# Autodesk Inventor assembly: heater assembly_v5
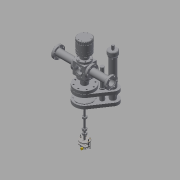
[picture p0: Inventor's stored thumbnail of the model, 180x180]
Saved by Autodesk Inventor 2019 (Build 230136000, 136)
## iProperties
Created: 2015-02-04
Part Number: heater assembly_v5
Document SubType Name: Assembly
Designer: Pascal
Author: Pascal
## Documents named in this file (13)
- C:\Users\user\Documents\Inventor@SVN\Moore Scienta DA30 system\e-beam-heater-Moore\heater assembly_v5.iam
- C:\Users\user\Documents\Inventor@SVN\Moore Scienta DA30 system\QMSC Heater_v3\rotary feedthrough (MDC 670024) length extension.ipt
- C:\Users\user\Documents\Inventor@SVN\Moore Scienta DA30 system\QMSC Heater_v3\9633T800_TWO-PIECE CLAMP-ON SHAFT COLLAR MOD.ipt
- C:\Users\user\Documents\Inventor@SVN\Moore Scienta DA30 system\QMSC Heater_v3\Ceramic eyelet.ipt
- C:\Users\user\Documents\Inventor@SVN\Moore Scienta DA30 system\QMSC Heater_v3\ANSI B18.2.2 - 6 - 32(06).ipt
- C:\Users\user\Documents\Inventor@SVN\Moore Scienta DA30 system\QMSC Heater_v3\MolyRodLong.ipt
- C:\Users\user\Documents\Inventor@SVN\Moore Scienta DA30 system\QMSC Heater_v3\BulletHolderAssembly.iam
- C:\Users\user\Documents\Inventor@SVN\Moore Scienta DA30 system\QMSC Heater_v3\MolyRodBulletPotential_v5.ipt
- C:\Users\user\Documents\Inventor@SVN\Moore Scienta DA30 system\QMSC Heater_v3\Shield_3_v5.ipt
- C:\Users\user\Documents\Inventor@SVN\Moore Scienta DA30 system\QMSC Heater_v3\2p75_6_way_cube_408001.ipt
- C:\Users\user\Documents\Inventor@SVN\Moore Scienta DA30 system\QMSC Heater_v3\4p5_to_2p75_reducer_402013.ipt
- C:\Users\user\Documents\Inventor@SVN\RM 479 ARPES and MOORE lab\diff_pump_stage\2p75_nipple_402002.ipt
- C:\Users\user\Documents\Inventor@SVN\Moore Scienta DA30 system\450LinearStage.iam
## Components (27 placed, 12 different names)
1. rotary feedthrough (MDC 670024) length extension:1 — Mate:45, Mate:47, Mate:49, Mate:53, Mate:111, Mate:162, Mate:171, Mate:182, Mate:183, Mate:190
2. 9633T800_TWO-PIECE CLAMP-ON SHAFT COLLAR MOD:1 — Mate:45, Mate:176, Mate:177
3. 9633T800_TWO-PIECE CLAMP-ON SHAFT COLLAR MOD:2 — Mate:49, Mate:50
4. 9633T800_TWO-PIECE CLAMP-ON SHAFT COLLAR MOD:3 — Mate:47, Mate:50
5. Shield_3_v5:1 — Mate:53, Mate:55, Mate:57, Mate:58, Mate:59, Mate:60, Mate:70, Mate:151, Mate:157, Mate:159, Mate:163, Mate:171, Mate:176, Mate:178, Mate:190
6. Ceramic eyelet:1 — Mate:55, Mate:155, Mate:156, Mate:157
7. Ceramic eyelet:2 — Mate:57, Mate:58, Mate:78, Mate:83, Mate:85
8. Ceramic eyelet:3 — Mate:59, Mate:60, Mate:61, Mate:62, Mate:63, Mate:64, Mate:161
9. Hex Machine Screw Nut - Inch 6 - 32:1 — Mate:61, Mate:62
10. Hex Machine Screw Nut - Inch 6 - 32:2 — Mate:63, Mate:64, Mate:174
11. Ceramic eyelet:7 — Mate:70, Flush:23, Mate:159, Mate:160
12. MolyRodBulletPotential_v5:1 — Mate:78, Mate:84, Mate:86, Flush:26, Mate:169
13. Hex Machine Screw Nut - Inch 6 - 32:3 — Mate:173, Mate:174, Mate:175
14. Hex Machine Screw Nut - Inch 6 - 32:4 — Mate:172, Mate:175
15. Hex Machine Screw Nut - Inch 6 - 32:5 — Mate:83, Mate:84
16. Hex Machine Screw Nut - Inch 6 - 32:6 — Mate:85, Mate:86
17. MolyRodBulletPotential_v5:2 — Mate:155, Mate:156, Flush:25, Mate:167
18. Hex Machine Screw Nut - Inch 6 - 32:7 — Mate:166, Mate:167
19. Hex Machine Screw Nut - Inch 6 - 32:8 — Mate:168, Mate:169
20. MolyRodLong:1 — Flush:24, Mate:160
21. MolyRodLong:2 — Flush:23, Flush:24, Mate:161, Mate:172, Mate:173
22. BulletHolderAssembly:1 [sub-assembly] — Mate:151, Flush:25, Flush:26, Mate:166, Mate:168, Mate:178, Mate:179, Angle:1
23. 2p75_6_way_cube_408001:1 — Mate:182, Mate:183, Mate:184, Mate:185, Mate:186, Mate:187
24. 4p5_to_2p75_reducer_402013:1 — Mate:188, Mate:189
25. 2p75_nipple_402002:1 — Mate:184, Mate:185
26. 2p75_nipple_402002:2 — Mate:186, Mate:187, Angle:1
27. 450LinearStage:1 [sub-assembly] — Mate:188, Mate:189
## Relationships (59: Mate 54, Flush 4, Angle 1)
- Mate:45: rotary feedthrough (MDC 670024) length extension:1 ↔ 9633T800_TWO-PIECE CLAMP-ON SHAFT COLLAR MOD:1
- Mate:47: rotary feedthrough (MDC 670024) length extension:1 ↔ 9633T800_TWO-PIECE CLAMP-ON SHAFT COLLAR MOD:3
- Mate:49: rotary feedthrough (MDC 670024) length extension:1 ↔ 9633T800_TWO-PIECE CLAMP-ON SHAFT COLLAR MOD:2
- Mate:50 (50.8 mm): 9633T800_TWO-PIECE CLAMP-ON SHAFT COLLAR MOD:2 ↔ 9633T800_TWO-PIECE CLAMP-ON SHAFT COLLAR MOD:3
- Mate:53: rotary feedthrough (MDC 670024) length extension:1 ↔ Shield_3_v5:1
- Mate:55: Shield_3_v5:1 ↔ Ceramic eyelet:1
- Mate:57: Shield_3_v5:1 ↔ Ceramic eyelet:2
- Mate:58: Shield_3_v5:1 ↔ Ceramic eyelet:2
- Mate:59: Shield_3_v5:1 ↔ Ceramic eyelet:3
- Mate:60: Shield_3_v5:1 ↔ Ceramic eyelet:3
- Mate:61: Ceramic eyelet:3 ↔ Hex Machine Screw Nut - Inch 6 - 32:1
- Mate:62: Ceramic eyelet:3 ↔ Hex Machine Screw Nut - Inch 6 - 32:1
- Mate:63: Ceramic eyelet:3 ↔ Hex Machine Screw Nut - Inch 6 - 32:2
- Mate:64: Ceramic eyelet:3 ↔ Hex Machine Screw Nut - Inch 6 - 32:2
- Mate:70: Shield_3_v5:1 ↔ Ceramic eyelet:7
- Mate:78: Ceramic eyelet:2 ↔ MolyRodBulletPotential_v5:1
- Mate:83: Ceramic eyelet:2 ↔ Hex Machine Screw Nut - Inch 6 - 32:5
- Mate:84: MolyRodBulletPotential_v5:1 ↔ Hex Machine Screw Nut - Inch 6 - 32:5
- Mate:85: Ceramic eyelet:2 ↔ Hex Machine Screw Nut - Inch 6 - 32:6
- Mate:86: MolyRodBulletPotential_v5:1 ↔ Hex Machine Screw Nut - Inch 6 - 32:6
- Flush:23 (-5.08 mm): Ceramic eyelet:7 ↔ MolyRodLong:2
- Flush:24: MolyRodLong:1 ↔ MolyRodLong:2
- Mate:111: rotary feedthrough (MDC 670024) length extension:1
- Mate:151 (19.05 mm): Shield_3_v5:1 ↔ BulletHolderAssembly:1
- Mate:155: Ceramic eyelet:1 ↔ MolyRodBulletPotential_v5:2
- Mate:156: Ceramic eyelet:1 ↔ MolyRodBulletPotential_v5:2
- Mate:157: Shield_3_v5:1 ↔ Ceramic eyelet:1
- Mate:159: Shield_3_v5:1 ↔ Ceramic eyelet:7
- Mate:160: Ceramic eyelet:7 ↔ MolyRodLong:1
- Mate:161: Ceramic eyelet:3 ↔ MolyRodLong:2
- Mate:162: rotary feedthrough (MDC 670024) length extension:1
- Mate:163: Shield_3_v5:1
- Flush:25: MolyRodBulletPotential_v5:2 ↔ BulletHolderAssembly:1
- Flush:26: MolyRodBulletPotential_v5:1 ↔ BulletHolderAssembly:1
- Mate:166: Hex Machine Screw Nut - Inch 6 - 32:7 ↔ BulletHolderAssembly:1
- Mate:167: MolyRodBulletPotential_v5:2 ↔ Hex Machine Screw Nut - Inch 6 - 32:7
- Mate:168: Hex Machine Screw Nut - Inch 6 - 32:8 ↔ BulletHolderAssembly:1
- Mate:169: MolyRodBulletPotential_v5:1 ↔ Hex Machine Screw Nut - Inch 6 - 32:8
- Mate:171: rotary feedthrough (MDC 670024) length extension:1 ↔ Shield_3_v5:1
- Mate:172: Hex Machine Screw Nut - Inch 6 - 32:4 ↔ MolyRodLong:2
- Mate:173: Hex Machine Screw Nut - Inch 6 - 32:3 ↔ MolyRodLong:2
- Mate:174 (38.1 mm): Hex Machine Screw Nut - Inch 6 - 32:2 ↔ Hex Machine Screw Nut - Inch 6 - 32:3
- Mate:175: Hex Machine Screw Nut - Inch 6 - 32:3 ↔ Hex Machine Screw Nut - Inch 6 - 32:4
- Mate:176 (25.4 mm): 9633T800_TWO-PIECE CLAMP-ON SHAFT COLLAR MOD:1 ↔ Shield_3_v5:1
- Mate:177: 9633T800_TWO-PIECE CLAMP-ON SHAFT COLLAR MOD:1
- Mate:178: Shield_3_v5:1 ↔ BulletHolderAssembly:1
- Mate:179: BulletHolderAssembly:1
- [Mate]: 2p75_6_way_cube_408001:1 ↔ 4p5_to_2p75_reducer_402013:1
- [Mate]: 2p75_6_way_cube_408001:1 ↔ 4p5_to_2p75_reducer_402013:1
- Mate:182: rotary feedthrough (MDC 670024) length extension:1 ↔ 2p75_6_way_cube_408001:1
- Mate:183: rotary feedthrough (MDC 670024) length extension:1 ↔ 2p75_6_way_cube_408001:1
- Mate:184: 2p75_6_way_cube_408001:1 ↔ 2p75_nipple_402002:1
- Mate:185: 2p75_6_way_cube_408001:1 ↔ 2p75_nipple_402002:1
- Mate:186: 2p75_6_way_cube_408001:1 ↔ 2p75_nipple_402002:2
- Mate:187: 2p75_6_way_cube_408001:1 ↔ 2p75_nipple_402002:2
- Mate:188: 4p5_to_2p75_reducer_402013:1 ↔ 450LinearStage:1
- Mate:189: 4p5_to_2p75_reducer_402013:1 ↔ 450LinearStage:1
- Mate:190: rotary feedthrough (MDC 670024) length extension:1 ↔ Shield_3_v5:1
- Angle:1 (90 deg): BulletHolderAssembly:1 ↔ 2p75_nipple_402002:2
